# Autodesk Inventor assembly: Z belt Sub
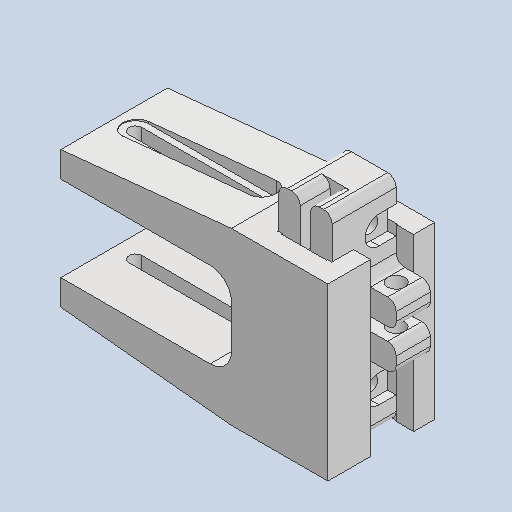
[picture p0: Inventor's stored thumbnail of the model, 512x512]
Saved by Autodesk Inventor 2022 (Build 260153000, 153)
## iProperties
Created: 2022-02-24
Part Number: Z belt Sub
Document SubType Name: Assembly
Designer: Nicoli
Author: Nicoli
## Documents named in this file (4)
- Y:\Projects\Bibble0\Z belt Sub.iam
- Y:\Projects\Bibble0\3D printed\Z Belt Clip.ipt
- Y:\Projects\Bibble0\Z Belt 2.ipt
- Y:\Projects\Bibble0\Z Belt 3.ipt
## Components (3 placed, 3 different names)
1. Z Belt Clip:1 — Insert:1, Insert:2, Mate:3
2. Z Belt 2:1 — Mate:2, Insert:1, Mate:3
3. Z Belt 3:1 — Mate:2, Insert:2
## Relationships (4: Mate 2, Insert 2)
- Mate:2: Z Belt 2:1 ↔ Z Belt 3:1
- Insert:1: Z Belt Clip:1 ↔ Z Belt 2:1
- Insert:2 (3 mm): Z Belt Clip:1 ↔ Z Belt 3:1
- Mate:3: Z Belt Clip:1 ↔ Z Belt 2:1
